# Autodesk Inventor assembly: leg_motor_moudle
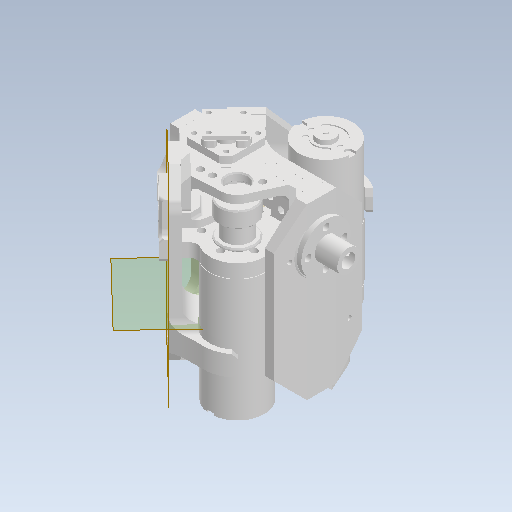
[picture p0: Inventor's stored thumbnail of the model, 512x512]
Saved by Autodesk Inventor 2020 (Build 240168000, 168)
## iProperties
Created: 2019-05-09
Part Number: leg_motor_moudle
Document SubType Name: Assembly
Designer: psrob
Author: psrob
## Documents named in this file (18)
- E:\projects-2\project dog gen2\hardware\leg_motor_moudle.iam
- E:\projects-2\project dog gen2\hardware\leg_basket_1.ipt
- E:\projects-2\project dog gen2\hardware\leg_basket_2.ipt
- E:\projects-2\project dog gen2\hardware\motor_holder.ipt
- E:\projects-2\project dog gen2\hardware\leg_basket_3.ipt
- E:\projects-2\project dog gen2\hardware\motor_2.ipt
- E:\projects-2\project dog gen2\hardware\pin_6_20.ipt
- E:\projects-2\project dog gen2\hardware\pin_6_60.ipt
- E:\projects-2\project dog gen2\hardware\2GT_wheel.ipt
- E:\projects-2\project dog gen2\hardware\bearing_6_13_5.ipt
- E:\projects-2\project dog gen2\hardware\flange_6mm.ipt
- E:\projects-2\project dog gen2\hardware\cross_axis_holder_1.ipt
- E:\projects-2\project dog gen2\hardware\2GT_wheel_5.ipt
- E:\projects-2\project dog gen2\hardware\encoder_ma1.ipt
- E:\projects-2\project dog gen2\hardware\encoder_ass.iam
- E:\projects-2\project dog gen2\hardware\belt_holder_2.ipt
- E:\projects-2\project dog gen2\hardware\motor_belt_wheel\timing-pulley-gt2-16-teeth-5mm-bore-2.snapshot.7\GT2-16T\GT2_16T.ipt
- E:\projects-2\project dog gen2\hardware\belt_pos_holder1.ipt
## Components (27 placed, 17 different names)
1. leg_basket_1:1 — Insert:1, Insert:2, Insert:3, Insert:4, Insert:5, Insert:6, Insert:7, Insert:8, Insert:28, Insert:29
2. leg_basket_2:1 — Insert:5, Insert:6, Insert:9, Insert:12, Insert:24, Insert:26, Insert:48, Insert:49, Insert:57
3. leg_basket_2:2 — Insert:7, Insert:8, Insert:10, Insert:11, Insert:25, Mate:1, Tangent:2, Insert:27, Insert:46, Insert:47, Insert:58
4. motor_holder:1 — Insert:1, Insert:2, Insert:19, Insert:20, Insert:56
5. motor_holder:2 — Insert:3, Insert:4, Insert:17, Insert:18
6. leg_basket_3:1 — Insert:11, Insert:12, Flush:1, Insert:54, Insert:55, Insert:59
7. leg_basket_3:2 — Insert:9, Insert:10, Insert:50, Insert:51
8. motor_2:1 — Insert:19, Insert:20
9. motor_2:2 — Insert:17, Insert:18, Insert:31
10. pin_6_20:1 — Insert:45
11. pin_6_60:1 — Tangent:1, Insert:44
12. 2GT_wheel:1
13. bearing_6_13_5:1 — Insert:24
14. bearing_6_13_5:2 — Insert:25
15. flange_6mm:1 — Mate:1, Tangent:1, Tangent:2
16. cross_axis_holder_1:1 — Insert:26, Insert:27, Flush:1
17. flange_6mm:2 — Insert:28, Insert:29
18. 2GT_wheel_5:1 — Insert:31
19. encoder_ma1:1 — Insert:44
20. encoder_ma1:2 — Insert:45
21. encoder_ass:1 [sub-assembly] — Insert:46, Insert:47
22. encoder_ass:2 [sub-assembly] — Insert:48, Insert:49
23. belt_holder_2:1 — Insert:50, Insert:51
24. belt_holder_2:2 — Insert:54, Insert:55
25. GT2_16T:1 — Insert:56, Flush:2
26. belt_pos_holder1:1 — Flush:2, Insert:57
27. belt_pos_holder1:2 — Insert:58, Insert:59
## Relationships (45: Insert 40, Tangent 2, Flush 2, Mate 1)
- Insert:1: leg_basket_1:1 ↔ motor_holder:1
- Insert:2: leg_basket_1:1 ↔ motor_holder:1
- Insert:3: leg_basket_1:1 ↔ motor_holder:2
- Insert:4: leg_basket_1:1 ↔ motor_holder:2
- Insert:5: leg_basket_1:1 ↔ leg_basket_2:1
- Insert:6: leg_basket_1:1 ↔ leg_basket_2:1
- Insert:7: leg_basket_1:1 ↔ leg_basket_2:2
- Insert:8: leg_basket_1:1 ↔ leg_basket_2:2
- Insert:9: leg_basket_2:1 ↔ leg_basket_3:2
- Insert:10: leg_basket_2:2 ↔ leg_basket_3:2
- Insert:11: leg_basket_2:2 ↔ leg_basket_3:1
- Insert:12: leg_basket_2:1 ↔ leg_basket_3:1
- Insert:17: motor_holder:2 ↔ motor_2:2
- Insert:18: motor_holder:2 ↔ motor_2:2
- Insert:19: motor_holder:1 ↔ motor_2:1
- Insert:20: motor_holder:1 ↔ motor_2:1
- [Insert] (-21 mm): pin_6_60:1 ↔ 2GT_wheel:1
- [Insert]: pin_6_20:1 ↔ bearing_6_13_5:1
- [Insert]: pin_6_60:1 ↔ bearing_6_13_5:2
- Insert:24: leg_basket_2:1 ↔ bearing_6_13_5:1
- Insert:25: leg_basket_2:2 ↔ bearing_6_13_5:2
- Mate:1 (-5 mm): leg_basket_2:2 ↔ flange_6mm:1
- Tangent:1: pin_6_60:1 ↔ flange_6mm:1
- Tangent:2: leg_basket_2:2 ↔ flange_6mm:1
- Insert:26: leg_basket_2:1 ↔ cross_axis_holder_1:1
- Insert:27: leg_basket_2:2 ↔ cross_axis_holder_1:1
- Flush:1: leg_basket_3:1 ↔ cross_axis_holder_1:1
- Insert:28: leg_basket_1:1 ↔ flange_6mm:2
- Insert:29: leg_basket_1:1 ↔ flange_6mm:2
- Insert:31 (-3 mm): motor_2:2 ↔ 2GT_wheel_5:1
- Insert:44: pin_6_60:1 ↔ encoder_ma1:1
- Insert:45: pin_6_20:1 ↔ encoder_ma1:2
- Insert:46: leg_basket_2:2 ↔ encoder_ass:1
- Insert:47: leg_basket_2:2 ↔ encoder_ass:1
- Insert:48: leg_basket_2:1 ↔ encoder_ass:2
- Insert:49: leg_basket_2:1 ↔ encoder_ass:2
- Insert:50: leg_basket_3:2 ↔ belt_holder_2:1
- Insert:51: leg_basket_3:2 ↔ belt_holder_2:1
- Insert:54: leg_basket_3:1 ↔ belt_holder_2:2
- Insert:55: leg_basket_3:1 ↔ belt_holder_2:2
- Insert:56 (2 mm): motor_holder:1 ↔ GT2_16T:1
- Flush:2: GT2_16T:1 ↔ belt_pos_holder1:1
- Insert:57: leg_basket_2:1 ↔ belt_pos_holder1:1
- Insert:58: leg_basket_2:2 ↔ belt_pos_holder1:2
- Insert:59: leg_basket_3:1 ↔ belt_pos_holder1:2
## Named parameters: d20_d12 = -21 mm
